# Autodesk Inventor assembly: Stewart-Platform-Base
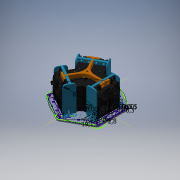
[picture p0: Inventor's stored thumbnail of the model, 180x180]
Saved by Autodesk Inventor 2018.2 (Build 222227000, 227)
## iProperties
Created: 2018-02-24
Part Number: Stewart-Platform-Base
Material: Generisch
Document SubType Name: Assembly
Designer: JochenAlt
Author: JochenAlt
## Documents named in this file (3)
- D:\Projects\Donna\CAD\Stewart-Platform-Base.iam
- D:\Projects\Donna\CAD\Stewart-Platform-Base.ipt
- D:\Projects\Donna\CAD\Servo-Holder.iam
## Components (4 placed, 2 different names)
1. Stewart-Platform-Base:1 — Passend:1, Passend:2, Passend:3, Passend:4, Passend:5, Passend:6, Passend:7, Passend:8, Passend:9, Passend:10
2. ServoHolder:1 [sub-assembly] — Passend:1, Passend:2
3. ServoHolder:2 [sub-assembly] — Passend:3, Passend:4
4. ServoHolder:3 [sub-assembly] — Passend:5, Passend:6
## Relationships (10: Mate 10)
- Passend:1 [Mate]: Stewart-Platform-Base:1 ↔ ServoHolder:1
- Passend:2 [Mate]: Stewart-Platform-Base:1 ↔ ServoHolder:1
- Passend:3 [Mate]: Stewart-Platform-Base:1 ↔ ServoHolder:2
- Passend:4 [Mate]: Stewart-Platform-Base:1 ↔ ServoHolder:2
- Passend:5 [Mate]: Stewart-Platform-Base:1 ↔ ServoHolder:3
- Passend:6 [Mate]: Stewart-Platform-Base:1 ↔ ServoHolder:3
- Passend:7 [Mate]: Stewart-Platform-Base:1
- Passend:8 [Mate]: Stewart-Platform-Base:1
- Passend:9 [Mate]: Stewart-Platform-Base:1
- Passend:10 [Mate]: Stewart-Platform-Base:1
